# Autodesk Inventor assembly: IR Sensor Mount
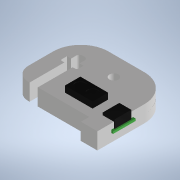
[picture p0: Inventor's stored thumbnail of the model, 180x180]
Saved by Autodesk Inventor 2020 (Build 240168000, 168)
## iProperties
Created: 2022-09-30
Part Number: IR Sensor Mount
Document SubType Name: Assembly
Designer: jsp534
Author: jsp534
## Documents named in this file (4)
- C:\Users\jsp534\OneDrive - University of York\Documents\_Projects\IR Sensor Mount\IR Sensor Mount.iam
- C:\Users\jsp534\OneDrive - University of York\Documents\_Projects\IR Sensor Mount\Front.ipt
- C:\Users\jsp534\OneDrive - University of York\Documents\_Projects\IR Sensor Mount\Back.ipt
- C:\Users\jsp534\OneDrive - University of York\Documents\_Projects\IR Sensor Mount\IR Sensor.ipt
## Components (3 placed, 3 different names)
1. Front:1 — Mate:2, Mate:3
2. Back:1 — Mate:1
3. IR Sensor:1 — Mate:1, Mate:2, Mate:3
## Relationships (3: Mate 3)
- Mate:1: Back:1 ↔ IR Sensor:1
- Mate:2 (0.1 mm): Front:1 ↔ IR Sensor:1
- Mate:3 (0.01 mm): Front:1 ↔ IR Sensor:1
